# Autodesk Inventor assembly: gate_and
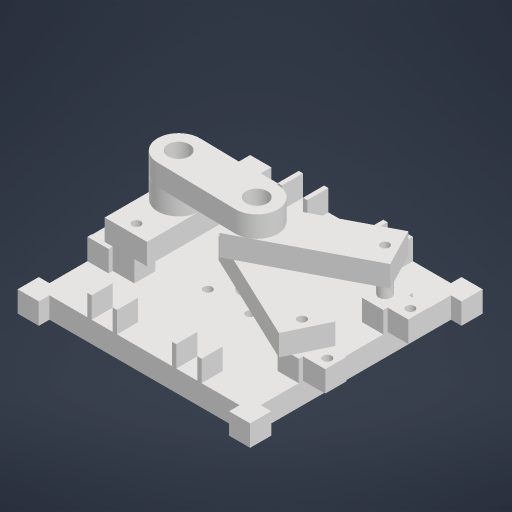
[picture p0: Inventor's stored thumbnail of the model, 512x512]
Saved by Autodesk Inventor 2024.3 (Build 283343000, 343)
## iProperties
Created: 2024-09-28
Part Number: gate_and
Document SubType Name: Assembly
Designer: sam
Author: sam
## Documents named in this file (8)
- N:\Cad\computer\gates\gate_and.iam
- N:\Cad\computer\gates\base.ipt
- N:\Cad\computer\gates\block.ipt
- N:\Cad\computer\gates\link_small.ipt
- N:\Cad\computer\gates\spacer_small.ipt
- N:\Cad\computer\gates\bar.ipt
- N:\Cad\computer\gates\connector.ipt
- N:\Cad\computer\gates\spacer.ipt
## Components (10 placed, 7 different names)
1. base:1 — Mate:1, Mate:2, Mate:3, Mate:4, Mate:5, Mate:6
2. block:1 — Mate:1, Mate:2, Mate:9, Mate:10
3. block:2 — Mate:3, Mate:4, Mate:7, Mate:8
4. block:3 — Mate:5, Mate:6, Mate:14, Mate:15, Flush:1
5. link_small:1 — Mate:11, Mate:12, Mate:13, Mate:17, Mate:18
6. link_small:2 — Mate:7, Mate:8, Mate:13
7. spacer_small:1 — Mate:9, Mate:10, Mate:11, Mate:12
8. bar:1 — Mate:14, Mate:15, Flush:1, Mate:16, Mate:20
9. connector:1 — Mate:16, Mate:17, Mate:18, Mate:19, Mate:21
10. spacer:1 — Mate:19, Mate:20, Mate:21
## Relationships (22: Mate 21, Flush 1)
- Mate:1: base:1 ↔ block:1
- Mate:2: base:1 ↔ block:1
- Mate:3: base:1 ↔ block:2
- Mate:4: base:1 ↔ block:2
- Mate:5: base:1 ↔ block:3
- Mate:6: base:1 ↔ block:3
- Mate:7: block:2 ↔ link_small:2
- Mate:8: block:2 ↔ link_small:2
- Mate:9: block:1 ↔ spacer_small:1
- Mate:10: block:1 ↔ spacer_small:1
- Mate:11: link_small:1 ↔ spacer_small:1
- Mate:12: link_small:1 ↔ spacer_small:1
- Mate:13: link_small:1 ↔ link_small:2
- Mate:14: block:3 ↔ bar:1
- Mate:15: block:3 ↔ bar:1
- Flush:1: block:3 ↔ bar:1
- Mate:16: bar:1 ↔ connector:1
- Mate:17: link_small:1 ↔ connector:1
- Mate:18: link_small:1 ↔ connector:1
- Mate:19: connector:1 ↔ spacer:1
- Mate:20: bar:1 ↔ spacer:1
- Mate:21: connector:1 ↔ spacer:1
